# Autodesk Inventor assembly: xs618b1mal2
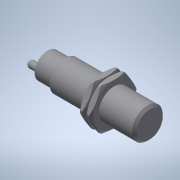
[picture p0: Inventor's stored thumbnail of the model, 180x180]
Saved by Autodesk Inventor 2021 (Build 250183000, 183)
## iProperties
Created: 2021-08-02
Part Number: xs618b1mal2
Checked By: TraceParts S.A.
Catalog Web Link: www.traceparts.com
Document SubType Name: Assembly
Designer: TraceParts
Company: TraceParts S.A.
SUPPLIER_NAME: RS Components
SUPPLIER: Schneider
DESIGN: Sensor inductivo, 8 mm, Salida NO, Cuerpo Cilíndrico, Rosca M18 x 1, 200 (dc) mA, 300 (ac) mA, 20 264 V ac/dc, IP69K
REFERENCE: XS618B1MAL2
Buy_Now: https://uk.rs-online.com/web/p/products/4443344?cm_mmc=en-ds-_-mcad-_-traceparts-_-4443344'
rs_stock_number: 4443344
TraceParts.PartVersion: 1.2.4
TraceParts.PartStatus: Published
TraceParts.PartNumber: 10-23062010-146802
TraceParts.PartLanguage: es
TraceParts.InstanceId: 10-23062010-14680214GR8C5PS4GPGYLPS7J4QJMIU
TraceParts.PartTitle: Sensor inductivo, 8 mm, Salida NO, Cuerpo Cilíndrico, Rosca M18 x 1, 200 (dc) mA, 300 (ac) mA, 20 264 V ac/dc, IP69K
TRACEPARTS: TRACEPARTS
TraceParts.ClassPath: RS_COMPONENTS:10-23062010-146802
Author: TraceParts
## Documents named in this file (4)
- D:\Nelson\Documentos\Inventor\Estacion_BocaPescado\xs618b1mal2.iam
- D:\Nelson\Documentos\Inventor\Estacion_BocaPescado\xs618b1mal2_01.ipt
- D:\Nelson\Documentos\Inventor\Estacion_BocaPescado\xs618b1mal2_02.ipt
- D:\Nelson\Documentos\Inventor\Estacion_BocaPescado\xs618b1mal2_03.ipt
## Components (3 placed, 3 different names)
1. xs618b1mal2_01:1 — Mate:1
2. xs618b1mal2_03:1 — Mate:2
3. xs618b1mal2_02:1 — Mate:1, Mate:2
## Relationships (2: Mate 2)
- Mate:1: xs618b1mal2_01:1 ↔ xs618b1mal2_02:1
- Mate:2 (0.9 mm): xs618b1mal2_03:1 ↔ xs618b1mal2_02:1
